# Autodesk Inventor assembly: Elevator Sprocket with Sprockets
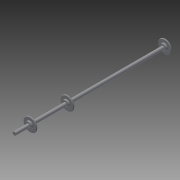
[picture p0: Inventor's stored thumbnail of the model, 180x180]
Saved by Autodesk Inventor 2015 (Build 190159000, 159)
## iProperties
Created: 2015-01-17
Part Number: Elevator Sprocket with Sprockets
Document SubType Name: Assembly
Designer: chapale16
Author: chapale16
## Documents named in this file (3)
- H:\Elevator Sprocket with Sprockets.iam
- H:\Elevator Axle.ipt
- H:\Sprocket Large.ipt
## Components (4 placed, 2 different names)
1. Elevator Axle:1 — Mate:1, Flush:1, Mate:2, Mate:3, Flush:3
2. Sprocket Large:1 — Mate:1, Flush:1, Flush:2, Flush:3
3. Sprocket Large:2 — Flush:2, Mate:2, Mate:4
4. Sprocket Large:3 — Mate:3, Mate:4
## Relationships (7: Mate 4, Flush 3)
- Mate:1: Elevator Axle:1 ↔ Sprocket Large:1
- Flush:1: Elevator Axle:1 ↔ Sprocket Large:1
- Flush:2 (361.95 mm): Sprocket Large:1 ↔ Sprocket Large:2
- Mate:2: Elevator Axle:1 ↔ Sprocket Large:2
- Mate:3: Elevator Axle:1 ↔ Sprocket Large:3
- Mate:4 (127 mm): Sprocket Large:2 ↔ Sprocket Large:3
- Flush:3: Elevator Axle:1 ↔ Sprocket Large:1
